# Autodesk Inventor assembly: !Structure
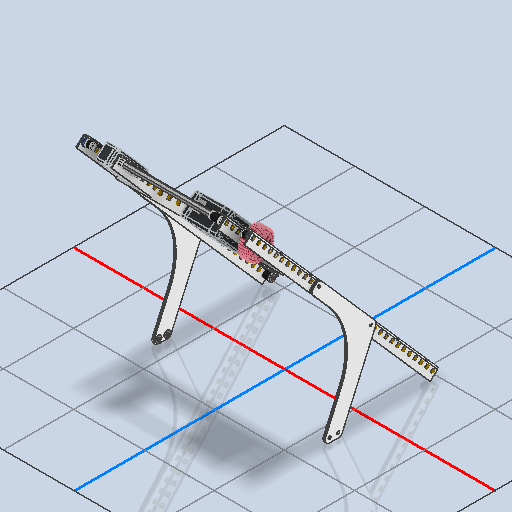
[picture p0: Inventor's stored thumbnail of the model, 512x512]
Saved by Autodesk Inventor 2026 (Build 300175000, 175)
## iProperties
Created: 2025-04-06
Part Number: !Structure
Document SubType Name: Assembly
Designer: avere
Author: avere
## Documents named in this file (26)
- C:\Users\avere\OneDrive\Documents\VEX-CAD\V5-CAD\Lady Brown\Structure\!Structure.iam
- C:\Users\avere\OneDrive\Documents\VEX-CAD\V5-CAD\Lady Brown\Structure\Custom Parts\Support Gusset.ipt
- C:\Users\avere\OneDrive\Documents\VEX-CAD\VEX-CAD-Inventor\Structure\C Channel\Aluminum 1x3x1 Half Thick Cut\Alu C Half Thick 1x3x1x32.ipt
- C:\Users\avere\OneDrive\Documents\VEX-CAD\VEX-CAD-Inventor\Structure\C Channel\Aluminum 1x3x1 Half Thick Cut\Alu C Half Thick 1x3x1x19.ipt
- C:\Users\avere\OneDrive\Documents\VEX-CAD\VEX-CAD-Inventor\Structure\C Channel\Aluminum 1x3x1 Half Thick Cut\Alu C Half Thick 1x3x1x8.ipt
- C:\Users\avere\OneDrive\Documents\VEX-CAD\VEX-CAD-Inventor\Electronics\Motors with Screws\SteelM-StarS.iam
- C:\Users\avere\OneDrive\Documents\VEX-CAD\VEX-CAD-Inventor\Electronics\Motors with Screws.iam
- C:\Users\avere\OneDrive\Documents\VEX-CAD\VEX-CAD-Inventor\Electronics\Sensors\V5 Rotation Sensor.ipt
- C:\Users\avere\OneDrive\Documents\VEX-CAD\VEX-CAD-Inventor\Motion\Spacers\Spacer Nylon .375 OD\NSpacer .375 OD x .375.ipt
- C:\Users\avere\OneDrive\Documents\VEX-CAD\VEX-CAD-Inventor\Motion\Spacers\Spacer Nylon .375 OD.ipt
- C:\Users\avere\OneDrive\Documents\VEX-CAD\VEX-CAD-Inventor\Motion\Spacers\Washer Steel\SWasher .375 OD x .062500.ipt
- C:\Users\avere\OneDrive\Documents\VEX-CAD\VEX-CAD-Inventor\Motion\Spacers\Washer Steel.ipt
- C:\Users\avere\OneDrive\Documents\VEX-CAD\VEX-CAD-Inventor\Motion\Spacers\Washer Steel\SWasher .375 OD x .015625.ipt
- C:\Users\avere\OneDrive\Documents\VEX-CAD\VEX-CAD-Inventor\Motion\Gears\HS Gear\HS 36T Gear, No Insert.iam
- C:\Users\avere\OneDrive\Documents\VEX-CAD\VEX-CAD-Inventor\Motion\Gears\HS Gear.iam
- C:\Users\avere\OneDrive\Documents\VEX-CAD\VEX-CAD-Inventor\Motion\Spacers\Washer Steel\SWasher .375 OD x .031250.ipt
- C:\Users\avere\OneDrive\Documents\VEX-CAD\VEX-CAD-Inventor\Motion\Spacers\Spacer Nylon .375 OD\NSpacer .375 OD x .125.ipt
- C:\Users\avere\OneDrive\Documents\VEX-CAD\VEX-CAD-Inventor\Motion\Shaft LS\Shaft Collar Metal\Shaft Collar Set Screw.ipt
- C:\Users\avere\OneDrive\Documents\VEX-CAD\VEX-CAD-Inventor\Motion\Shaft LS\Bearing Flat Low Profile.ipt
- C:\Users\avere\OneDrive\Documents\VEX-CAD\VEX-CAD-Inventor\Motion\Spacers\Spacer Nylon .375 OD\NSpacer .375 OD x .250.ipt
- C:\Users\avere\OneDrive\Documents\VEX-CAD\VEX-CAD-Inventor\Structure\Standoff\Standoff 5.00.ipt
- C:\Users\avere\OneDrive\Documents\VEX-CAD\VEX-CAD-Inventor\Structure\Standoff.ipt
- C:\Users\avere\OneDrive\Documents\VEX-CAD\VEX-CAD-Inventor\Structure\Hardware\Nut Keps.ipt
- C:\Users\avere\OneDrive\Documents\VEX-CAD\VEX-CAD-Inventor\Motion\Spacers\Washer Teflon\TWasher .375 OD x .04000.ipt
- C:\Users\avere\OneDrive\Documents\VEX-CAD\VEX-CAD-Inventor\Motion\Spacers\Washer Teflon.ipt
- C:\Users\avere\OneDrive\Documents\VEX-CAD\VEX-CAD-Inventor\Motion\Spacers\Spacer Nylon .375 OD\NSpacer .375 OD x .500.ipt
## Components (38 placed, 19 different names)
1. Alu C Half Thick 1x3x1x32:1 — Mate:4, Angle:1, Mate:11, Mate:13, Insert:12, Insert:17, Insert:22, Mate:16, Insert:31
2. Support Gusset:1 — Insert:13, Insert:14
3. Support Gusset:2 — Mate:3, Mate:5
4. Alu C Half Thick 1x3x1x32:2 — Angle:2, Mate:6, Insert:3, Mate:7, Insert:5
5. Support Gusset:3 — Insert:3, Mate:7, Insert:4, Mate:10
6. Support Gusset:4 — Mate:8, Mate:9, Insert:4, Mate:10
7. Alu C Half Thick 1x3x1x19:1 — Insert:5, Mate:11, Insert:7, Insert:39
8. Alu C Half Thick 1x3x1x8:1 — Insert:7, Mate:13, Insert:24, Mate:17
9. SteelM-StarS:1 [sub-assembly]
10. Alu C Half Thick 1x3x1x8:2 — Insert:39, Insert:40, Mate:23, Insert:41, Mate:24
11. V5 Rotation Sensor:1 — Insert:40, Mate:23
12. NSpacer .375 OD x .375:1 — Insert:10, Insert:12
13. SWasher .375 OD x .062500:1 — Insert:10, Insert:11
14. SWasher .375 OD x .015625:2 — Insert:11
15. SWasher .375 OD x .015625:3 — Insert:14
16. SWasher .375 OD x .015625:4 — Insert:13
17. NSpacer .375 OD x .375:2 — Insert:15
18. SWasher .375 OD x .062500:5 — Insert:15, Insert:16
19. SWasher .375 OD x .015625:6 — Insert:16
20. SWasher .375 OD x .015625:7
21. SWasher .375 OD x .015625:8
22. HS 36T Gear, No Insert:1 [sub-assembly] — Insert:17, Insert:21
23. SWasher .375 OD x .031250:9 — Insert:19, Insert:20
24. SWasher .375 OD x .015625:10 — Insert:20
25. NSpacer .375 OD x .125:3 — Insert:18, Insert:19
26. Shaft Collar Set Screw:1 — Insert:18, Insert:21
27. Bearing Flat Low Profile:1 — Insert:22, Mate:16, Insert:23
28. NSpacer .375 OD x .250:4 — Insert:23
29. Bearing Flat Low Profile:2 — Insert:24, Mate:17
30. Nut Keps:1 — Insert:31, Insert:33
31. NSpacer .375 OD x .250:6 — Insert:32
32. TWasher .375 OD x .04000:1 — Insert:32, Insert:33
33. Nut Keps:2 — Insert:34
34. NSpacer .375 OD x .250:7 — Insert:35
35. TWasher .375 OD x .04000:2 — Insert:34, Insert:35
36. Bearing Flat Low Profile:3 — Insert:41, Mate:24, Insert:42
37. Standoff 5.00:1 — Insert:42, Insert:43
38. NSpacer .375 OD x .500:8 — Insert:43
## Relationships (51: Insert 32, Mate 17, Angle 2)
- [Insert]: Support Gusset:1 ↔ Support Gusset:2
- [Mate]: Support Gusset:1 ↔ Support Gusset:2
- [Insert]: Alu C Half Thick 1x3x1x32:1 ↔ Support Gusset:1
- [Mate]: Alu C Half Thick 1x3x1x32:1 ↔ Support Gusset:1
- Mate:3: Support Gusset:2
- Mate:4 (114.3 mm): Alu C Half Thick 1x3x1x32:1
- Angle:1 (0 deg): Alu C Half Thick 1x3x1x32:1
- Mate:5: Support Gusset:2
- Angle:2 (0 deg): Alu C Half Thick 1x3x1x32:2
- Mate:6 (-114.3 mm): Alu C Half Thick 1x3x1x32:2
- Insert:3: Alu C Half Thick 1x3x1x32:2 ↔ Support Gusset:3
- Mate:7: Alu C Half Thick 1x3x1x32:2 ↔ Support Gusset:3
- Mate:8: Support Gusset:4
- Mate:9: Support Gusset:4
- Insert:4: Support Gusset:3 ↔ Support Gusset:4
- Mate:10: Support Gusset:3 ↔ Support Gusset:4
- Insert:5: Alu C Half Thick 1x3x1x32:2 ↔ Alu C Half Thick 1x3x1x19:1
- Mate:11: Alu C Half Thick 1x3x1x32:1 ↔ Alu C Half Thick 1x3x1x19:1
- [Insert]: Alu C Half Thick 1x3x1x8:1 ↔ SteelM-StarS:1
- [Mate]: Alu C Half Thick 1x3x1x8:1 ↔ SteelM-StarS:1
- Insert:7: Alu C Half Thick 1x3x1x19:1 ↔ Alu C Half Thick 1x3x1x8:1
- Mate:13: Alu C Half Thick 1x3x1x32:1 ↔ Alu C Half Thick 1x3x1x8:1
- Insert:10: NSpacer .375 OD x .375:1 ↔ SWasher .375 OD x .062500:1
- Insert:11: SWasher .375 OD x .062500:1 ↔ SWasher .375 OD x .015625:2
- Insert:12: Alu C Half Thick 1x3x1x32:1 ↔ NSpacer .375 OD x .375:1
- Insert:13: Support Gusset:1 ↔ SWasher .375 OD x .015625:4
- Insert:14: Support Gusset:1 ↔ SWasher .375 OD x .015625:3
- Insert:15: NSpacer .375 OD x .375:2 ↔ SWasher .375 OD x .062500:5
- Insert:16: SWasher .375 OD x .062500:5 ↔ SWasher .375 OD x .015625:6
- Insert:17 (12.7 mm): Alu C Half Thick 1x3x1x32:1 ↔ HS 36T Gear, No Insert:1
- Insert:18: NSpacer .375 OD x .125:3 ↔ Shaft Collar Set Screw:1
- Insert:19: SWasher .375 OD x .031250:9 ↔ NSpacer .375 OD x .125:3
- Insert:20: SWasher .375 OD x .031250:9 ↔ SWasher .375 OD x .015625:10
- Insert:21: HS 36T Gear, No Insert:1 ↔ Shaft Collar Set Screw:1
- Insert:22: Alu C Half Thick 1x3x1x32:1 ↔ Bearing Flat Low Profile:1
- Mate:16: Alu C Half Thick 1x3x1x32:1 ↔ Bearing Flat Low Profile:1
- Insert:23 (1.27 mm): Bearing Flat Low Profile:1 ↔ NSpacer .375 OD x .250:4
- Insert:24: Alu C Half Thick 1x3x1x8:1 ↔ Bearing Flat Low Profile:2
- Mate:17: Alu C Half Thick 1x3x1x8:1 ↔ Bearing Flat Low Profile:2
- Insert:31: Alu C Half Thick 1x3x1x32:1 ↔ Nut Keps:1
- Insert:32: NSpacer .375 OD x .250:6 ↔ TWasher .375 OD x .04000:1
- Insert:33: Nut Keps:1 ↔ TWasher .375 OD x .04000:1
- Insert:34: Nut Keps:2 ↔ TWasher .375 OD x .04000:2
- Insert:35: NSpacer .375 OD x .250:7 ↔ TWasher .375 OD x .04000:2
- Insert:39: Alu C Half Thick 1x3x1x19:1 ↔ Alu C Half Thick 1x3x1x8:2
- Insert:40: Alu C Half Thick 1x3x1x8:2 ↔ V5 Rotation Sensor:1
- Mate:23: Alu C Half Thick 1x3x1x8:2 ↔ V5 Rotation Sensor:1
- Insert:41: Alu C Half Thick 1x3x1x8:2 ↔ Bearing Flat Low Profile:3
- Mate:24: Alu C Half Thick 1x3x1x8:2 ↔ Bearing Flat Low Profile:3
- Insert:42 (1.27 mm): Bearing Flat Low Profile:3 ↔ Standoff 5.00:1
- Insert:43: Standoff 5.00:1 ↔ NSpacer .375 OD x .500:8
